# Autodesk Inventor assembly: s-assy-link3
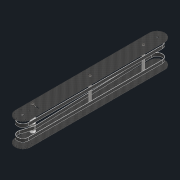
[picture p0: Inventor's stored thumbnail of the model, 180x180]
Saved by Autodesk Inventor 2021 (Build 250183000, 183)
## iProperties
Created: 2021-07-17
Part Number: s-assy-link3
Document SubType Name: Assembly
Designer: yuta0
Mass: 1448.61 g
Surface Area: 6046.34 cm^2
Volume: 815.942 cm^3
Density: 1.77539 g/cm^3
Author: yuta0
## Documents named in this file (5)
- C:\Users\yuta0\Desktop\catchrobo_robot\s-assy-link3.iam
- C:\Users\yuta0\Desktop\catchrobo_robot\carbon_plate4.ipt
- C:\Users\yuta0\Desktop\catchrobo_robot\belt_3.ipt
- C:\Users\yuta0\Desktop\catchrobo_robot\s-assy-spacer3.iam
- C:\Users\yuta0\Desktop\catchrobo_robot\s-assy-spacer1.iam
## Components (7 placed, 4 different names)
1. carbon_plate4:1 — フラッシュ:1, メイト:253, メイト:254, フラッシュ:3, メイト:262, メイト:263, メイト:264, メイト:269, メイト:270
2. carbon_plate4:2 — フラッシュ:1, メイト:254, メイト:261, メイト:265, メイト:266, メイト:267, メイト:268
3. belt_3:1 — メイト:252, メイト:258, メイト:267, メイト:268
4. belt_3:2 — メイト:259, メイト:269, メイト:270
5. s-assy-spacer3:1 [sub-assembly] — メイト:252, メイト:266, フラッシュ:4
6. s-assy-spacer1:1 [sub-assembly] — メイト:261, メイト:262, メイト:265
7. s-assy-spacer1:2 [sub-assembly] — メイト:263, メイト:264
## Relationships (18: Mate 15, Flush 3)
- フラッシュ:1 [Flush]: carbon_plate4:1 ↔ carbon_plate4:2
- メイト:252 [Mate]: belt_3:1 ↔ s-assy-spacer3:1
- メイト:253 [Mate]: carbon_plate4:1
- メイト:254 [Mate]: carbon_plate4:1 ↔ carbon_plate4:2
- メイト:258 [Mate]: belt_3:1
- メイト:259 [Mate]: belt_3:2
- フラッシュ:3 [Flush]: carbon_plate4:1
- メイト:261 [Mate]: carbon_plate4:2 ↔ s-assy-spacer1:1
- メイト:262 [Mate]: carbon_plate4:1 ↔ s-assy-spacer1:1
- メイト:263 [Mate]: carbon_plate4:1 ↔ s-assy-spacer1:2
- メイト:264 [Mate]: carbon_plate4:1 ↔ s-assy-spacer1:2
- メイト:265 [Mate]: carbon_plate4:2 ↔ s-assy-spacer1:1
- メイト:266 [Mate]: carbon_plate4:2 ↔ s-assy-spacer3:1
- メイト:267 [Mate] (12.15 mm): carbon_plate4:2 ↔ belt_3:1
- メイト:268 [Mate]: carbon_plate4:2 ↔ belt_3:1
- メイト:269 [Mate]: carbon_plate4:1 ↔ belt_3:2
- メイト:270 [Mate] (12.15 mm): carbon_plate4:1 ↔ belt_3:2
- フラッシュ:4 [Flush]: s-assy-spacer3:1
